# Autodesk Inventor assembly: S8x1
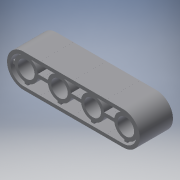
[picture p0: Inventor's stored thumbnail of the model, 180x180]
Saved by Autodesk Inventor 2019 (Build 230136000, 136)
## iProperties
Created: 2019-01-31
Part Number: S8x1
Document SubType Name: Assembly
Designer: Varga Daniel
Author: Varga Daniel
## Documents named in this file (3)
- C:\!_Dani\!_cloud\OneDrive\!_munka\Revolution\RevvyDemoKit\Structural parts\Straight Beams\S4x1.iam
- C:\!_Dani\!_cloud\OneDrive\!_munka\Revolution\RevvyDemoKit\Structural parts\Straight Beams\straight_beam_inner_part_single.ipt
- C:\!_Dani\!_cloud\OneDrive\!_munka\Revolution\RevvyDemoKit\Structural parts\Straight Beams\straight_beam_end_part_single.ipt
## Components (4 placed, 2 different names)
1. straight_beam_inner_part_single:1 — Mate:5, Flush:13, Flush:14, Mate:8
2. straight_beam_inner_part_single:2 — Mate:5, Flush:11, Flush:12, Mate:7
3. straight_beam_end_part_single:1 — Flush:13, Flush:14, Mate:8
4. straight_beam_end_part_single:2 — Flush:11, Flush:12, Mate:7
## Relationships (7: Flush 4, Mate 3)
- Mate:5: straight_beam_inner_part_single:1 ↔ straight_beam_inner_part_single:2
- Flush:11: straight_beam_inner_part_single:2 ↔ straight_beam_end_part_single:2
- Flush:12: straight_beam_inner_part_single:2 ↔ straight_beam_end_part_single:2
- Mate:7: straight_beam_inner_part_single:2 ↔ straight_beam_end_part_single:2
- Flush:13: straight_beam_inner_part_single:1 ↔ straight_beam_end_part_single:1
- Flush:14: straight_beam_inner_part_single:1 ↔ straight_beam_end_part_single:1
- Mate:8: straight_beam_inner_part_single:1 ↔ straight_beam_end_part_single:1
